# Autodesk Inventor assembly: CameraSetup
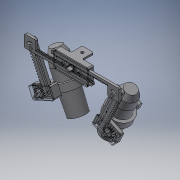
[picture p0: Inventor's stored thumbnail of the model, 180x180]
Saved by Autodesk Inventor 2019 (Build 230136000, 136)
## iProperties
Created: 2019-07-15
Part Number: CameraSetup
Document SubType Name: Assembly
Designer: aorfi
Author: aorfi
## Documents named in this file (13)
- C:\Users\aorfi\Documents\IQC\CameraSetup.iam
- C:\Users\aorfi\Documents\IQC\COTS\USBCamera.ipt
- C:\Users\aorfi\Documents\IQC\CustomParts\CameraClamp.ipt
- C:\Users\aorfi\Documents\IQC\CustomParts\Rack.ipt
- C:\Users\aorfi\Documents\IQC\CustomParts\Pinion.ipt
- C:\Users\aorfi\Documents\IQC\CustomParts\PinionHolder.ipt
- C:\Users\aorfi\Documents\IQC\CustomParts\GearCover.ipt
- C:\Users\aorfi\Documents\IQC\CustomParts\CameraBaseRight.ipt
- C:\Users\aorfi\Documents\IQC\CustomParts\CameraBaseLeft.ipt
- C:\Users\aorfi\Documents\IQC\CustomParts\CameraLinearSupporter.ipt
- C:\Users\aorfi\Documents\IQC\CustomParts\SmallPinion.ipt
- C:\Users\aorfi\Documents\IQC\CustomParts\RackMirror.ipt
- C:\Users\aorfi\Documents\IQC\CustomParts\GearCoverTop.ipt
## Components (17 placed, 12 different names)
1. USBCamera:2 — Mate:2, Symmetry:1, Mate:10
2. CameraClamp:1 — Mate:1, Symmetry:2, Mate:11, Mate:70, Mate:71, Mate:72
3. USBCamera:1 — Mate:1, Symmetry:1, Mate:11
4. CameraClamp:2 — Mate:2, Symmetry:2, Mate:10, Mate:24, Mate:25, Mate:36
5. Rack:1 — Mate:34, Mate:35, Mate:42, Mate:43, Mate:56
6. Pinion:1 — Mate:29, Mate:30
7. PinionHolder:1 — Mate:24, Mate:25, Mate:29, Mate:30, Mate:34, Mate:35, Mate:36, Mate:38, Mate:39, Mate:56, Mate:58
8. GearCover:1 — Mate:38, Mate:39, Mate:58
9. CameraBaseRight:1 — Mate:42, Mate:43, Mate:46, Mate:47, Symmetry:4
10. CameraBaseLeft:1 — Mate:50, Mate:51, Mate:53, Mate:54, Symmetry:4
11. CameraLinearSupporter:1 — Mate:46, Mate:47, Mate:48, Mate:49, Mate:50, Mate:51, Mate:55, Mate:57, Flush:1, Mate:59, Flush:2, Flush:3, Mate:60
12. SmallPinion:1 — Mate:55, Mate:60
13. RackMirror:1 — Mate:53, Mate:54, Mate:68, Mate:69
14. GearCoverTop:1 — Mate:59, Flush:2, Flush:3
15. PinionHolder:2 — Mate:63, Mate:64, Mate:65, Mate:66, Mate:67, Mate:68, Mate:69, Mate:70, Mate:71, Mate:72
16. GearCover:2 — Mate:65, Mate:66, Mate:67
17. Pinion:2 — Mate:63, Mate:64
## Relationships (45: Mate 39, Symmetry 3, Flush 3)
- Mate:1: CameraClamp:1 ↔ USBCamera:1
- Mate:2: USBCamera:2 ↔ CameraClamp:2
- Symmetry:1: USBCamera:2 ↔ USBCamera:1
- Symmetry:2: CameraClamp:1 ↔ CameraClamp:2
- Mate:10: USBCamera:2 ↔ CameraClamp:2
- Mate:11: CameraClamp:1 ↔ USBCamera:1
- Mate:24: CameraClamp:2 ↔ PinionHolder:1
- Mate:25: CameraClamp:2 ↔ PinionHolder:1
- Mate:29: Pinion:1 ↔ PinionHolder:1
- Mate:30: Pinion:1 ↔ PinionHolder:1
- Mate:34: Rack:1 ↔ PinionHolder:1
- Mate:35: Rack:1 ↔ PinionHolder:1
- Mate:36: CameraClamp:2 ↔ PinionHolder:1
- Mate:38: PinionHolder:1 ↔ GearCover:1
- Mate:39: PinionHolder:1 ↔ GearCover:1
- Mate:42: Rack:1 ↔ CameraBaseRight:1
- Mate:43: Rack:1 ↔ CameraBaseRight:1
- Mate:46: CameraBaseRight:1 ↔ CameraLinearSupporter:1
- Mate:47: CameraBaseRight:1 ↔ CameraLinearSupporter:1
- Mate:48: CameraLinearSupporter:1
- Mate:49: CameraLinearSupporter:1
- Mate:50: CameraBaseLeft:1 ↔ CameraLinearSupporter:1
- Mate:51: CameraBaseLeft:1 ↔ CameraLinearSupporter:1
- Mate:53: CameraBaseLeft:1 ↔ RackMirror:1
- Mate:54: CameraBaseLeft:1 ↔ RackMirror:1
- Mate:55: CameraLinearSupporter:1 ↔ SmallPinion:1
- Mate:56: Rack:1 ↔ PinionHolder:1
- Mate:57: CameraLinearSupporter:1
- Flush:1: CameraLinearSupporter:1
- Mate:58: PinionHolder:1 ↔ GearCover:1
- Symmetry:4: CameraBaseRight:1 ↔ CameraBaseLeft:1
- Mate:59: CameraLinearSupporter:1 ↔ GearCoverTop:1
- Flush:2: CameraLinearSupporter:1 ↔ GearCoverTop:1
- Flush:3: CameraLinearSupporter:1 ↔ GearCoverTop:1
- Mate:60: CameraLinearSupporter:1 ↔ SmallPinion:1
- Mate:63: PinionHolder:2 ↔ Pinion:2
- Mate:64: PinionHolder:2 ↔ Pinion:2
- Mate:65: PinionHolder:2 ↔ GearCover:2
- Mate:66: PinionHolder:2 ↔ GearCover:2
- Mate:67: PinionHolder:2 ↔ GearCover:2
- Mate:68: RackMirror:1 ↔ PinionHolder:2
- Mate:69: RackMirror:1 ↔ PinionHolder:2
- Mate:70: CameraClamp:1 ↔ PinionHolder:2
- Mate:71: CameraClamp:1 ↔ PinionHolder:2
- Mate:72: CameraClamp:1 ↔ PinionHolder:2
